# Autodesk Inventor assembly: Ensamblaje Prueba
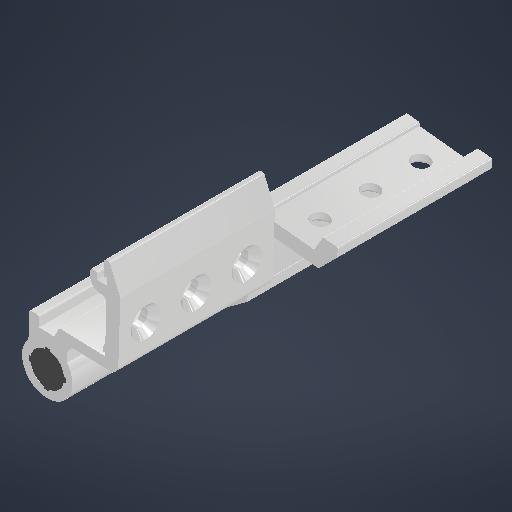
[picture p0: Inventor's stored thumbnail of the model, 512x512]
Saved by Autodesk Inventor 2025 (Build 290162000, 162)
## iProperties
Created: 2026-02-04
Part Number: Ensamblaje Prueba
Document SubType Name: Assembly
Designer: ROLANDO
Author: ROLANDO
## Documents named in this file (6)
- C:\Users\rolan\OneDrive\Documentos\Inventor\Projects\CARPINTERIA ALUMINIO\PUERTAS Y VENTANAS\BISAGRA\Ensamblaje Prueba.iam
- C:\Users\rolan\OneDrive\Documentos\Inventor\Projects\CARPINTERIA ALUMINIO\PUERTAS Y VENTANAS\BISAGRA\HIN-61 BISAGRA (P1).ipt
- HIN-61 BISAGRA (P1).ipt
- C:\Users\rolan\OneDrive\Documentos\Inventor\Projects\CARPINTERIA ALUMINIO\PUERTAS Y VENTANAS\BISAGRA\HIN-61 BISAGRA (P2).ipt
- C:\Users\rolan\OneDrive\Documentos\Inventor\Projects\CARPINTERIA ALUMINIO\PUERTAS Y VENTANAS\BISAGRA\HIN-61 BISAGRA (PASADOR).ipt
- C:\Users\rolan\OneDrive\Documentos\Inventor\Projects\CARPINTERIA ALUMINIO\PUERTAS Y VENTANAS\BISAGRA\HIN-61 BISAGRA (BUJE PLASTICO).ipt
## Components (5 placed, 3 different names)
1. HIN-61 BISAGRA (P1):1 — Coincidencia:1, Coincidencia:2, Coincidencia:3
2. HIN-61 BISAGRA (BUJE PLASTICO):1 — Coincidencia:1, Coincidencia:2, Coincidencia:3, Insertar:2
3. HIN-61 BISAGRA (P1):2 — Coincidencia:5, Coincidencia:6, Coincidencia:7
4. HIN-61 BISAGRA (BUJE PLASTICO):2 — Coincidencia:5, Coincidencia:6, Coincidencia:7, Insertar:1
5. HIN-61 BISAGRA (PASADOR):1 — Insertar:1, Insertar:2
## Relationships (8: Mate 6, Insert 2)
- Coincidencia:1 [Mate]: HIN-61 BISAGRA (P1):1 ↔ HIN-61 BISAGRA (BUJE PLASTICO):1
- Coincidencia:2 [Mate]: HIN-61 BISAGRA (P1):1 ↔ HIN-61 BISAGRA (BUJE PLASTICO):1
- Coincidencia:3 [Mate]: HIN-61 BISAGRA (P1):1 ↔ HIN-61 BISAGRA (BUJE PLASTICO):1
- Coincidencia:5 [Mate]: HIN-61 BISAGRA (P1):2 ↔ HIN-61 BISAGRA (BUJE PLASTICO):2
- Coincidencia:6 [Mate]: HIN-61 BISAGRA (P1):2 ↔ HIN-61 BISAGRA (BUJE PLASTICO):2
- Coincidencia:7 [Mate]: HIN-61 BISAGRA (P1):2 ↔ HIN-61 BISAGRA (BUJE PLASTICO):2
- Insertar:1 (-39.5 mm): HIN-61 BISAGRA (BUJE PLASTICO):2 ↔ HIN-61 BISAGRA (PASADOR):1
- Insertar:2 (-39.5 mm): HIN-61 BISAGRA (BUJE PLASTICO):1 ↔ HIN-61 BISAGRA (PASADOR):1
